# Autodesk Inventor assembly: Сборка1
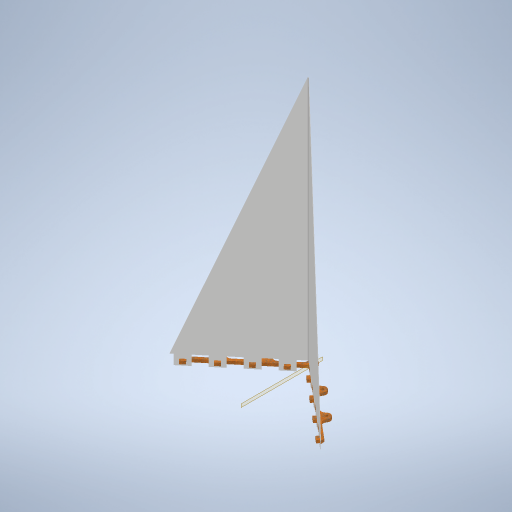
[picture p0: Inventor's stored thumbnail of the model, 512x512]
Saved by Autodesk Inventor 2023 (Build 270158000, 158)
## iProperties
Created: 2024-02-14
Part Number: Сборка1
Document SubType Name: Assembly
Designer: liza
Author: liza
## Documents named in this file (3)
- C:\Users\liza\Desktop\Work\Crow_Sborka\Сборка1.iam
- C:\Users\liza\Desktop\Work\Crow_Sborka\клюв.ipt
- C:\Users\liza\Desktop\Work\Crow_Sborka\крепежная деталь для клюва.ipt
## Components (2 placed, 2 different names)
1. клюв:1 — Совмещение:2, Совмещение:3, Совмещение:4
2. крепежная деталь для клюва:1 — Совмещение:2, Совмещение:3, Совмещение:4
## Relationships (3: Mate 3)
- Совмещение:2 [Mate]: клюв:1 ↔ крепежная деталь для клюва:1
- Совмещение:3 [Mate]: клюв:1 ↔ крепежная деталь для клюва:1
- Совмещение:4 [Mate]: клюв:1 ↔ крепежная деталь для клюва:1
